# Autodesk Inventor assembly: final assembly
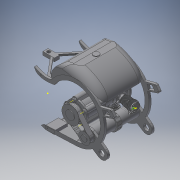
[picture p0: Inventor's stored thumbnail of the model, 180x180]
Saved by Autodesk Inventor 2018 (Build 220112000, 112)
## iProperties
Created: 2021-03-15
Part Number: final assembly
Document SubType Name: Assembly
Designer: Jyoti Soni
Author: Jyoti Soni
## Documents named in this file (4)
- C:\Users\Jyoti Soni\Desktop\asm\15032021\final assembly.iam
- C:\Users\Jyoti Soni\Downloads\Part2 new project.ipt
- C:\Users\Jyoti Soni\Desktop\asm\15032021\cylinder asm.iam
- C:\Users\Jyoti Soni\Desktop\chain sproket.ipt
## Components (3 placed, 3 different names)
1. Part2 new project:1 — Flush:1, Mate:1, Mate:2, Mate:3
2. cylinder asm:1 [sub-assembly] — Flush:1, Mate:2, Mate:5
3. chain sproket:1 — Mate:3, Mate:4, Mate:5
## Relationships (6: Mate 5, Flush 1)
- Flush:1 (-10 mm): Part2 new project:1 ↔ cylinder asm:1
- Mate:1: Part2 new project:1
- Mate:2: Part2 new project:1 ↔ cylinder asm:1
- Mate:3: Part2 new project:1 ↔ chain sproket:1
- Mate:4: chain sproket:1
- Mate:5 (10 mm): cylinder asm:1 ↔ chain sproket:1
